# Autodesk Inventor assembly: Pick_&_Place_Nozzle_Assembly
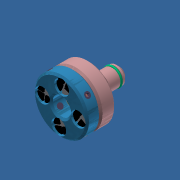
[picture p0: Inventor's stored thumbnail of the model, 180x180]
Saved by Autodesk Inventor 2015 (Build 190159000, 159)
## iProperties
Created: 2015-01-06
Part Number: Pick_&_Place_Nozzle_Assembly
Document SubType Name: Assembly
Designer: ice
Author: ice
## Documents named in this file (8)
- C:\Users\ice\Documents\GitHub\PnP-Magnetic-Tool-Tip\Inventor\Extender_Assembly_Rev_C.iam
- C:\Users\ice\Documents\GitHub\PnP-Magnetic-Tool-Tip\Inventor\Magnet_Extender_Split_Top_Rev_C.ipt
- C:\Users\ice\Documents\GitHub\PnP-Magnetic-Tool-Tip\Inventor\Magnet_Extender_Split_Bottom_Rev_C.ipt
- C:\Users\ice\Documents\GitHub\PnP-Magnetic-Tool-Tip\Inventor\o_ring_5.00_0.5.ipt
- C:\Users\ice\Documents\GitHub\PnP-Magnetic-Tool-Tip\Inventor\M1.6x5_Headless.ipt
- C:\Users\ice\Documents\GitHub\PnP-Magnetic-Tool-Tip\Inventor\M2x5_D963.ipt
- C:\Users\ice\Documents\GitHub\PnP-Magnetic-Tool-Tip\Inventor\o_ring_4.29_0.5XXX.ipt
- C:\Users\ice\Documents\GitHub\PnP-Magnetic-Tool-Tip\Inventor\Magnet10x1x5.ipt
## Components (14 placed, 7 different names)
1. Magnet_Extender_Split_Top_Rev_C:1 — Mate:1, Mate:2, Mate:3, Mate:5, Mate:20, Mate:21, Mate:22, Flush:3, Mate:23, Flush:4
2. Magnet_Extender_Split_Bottom_Rev_C:1 — Mate:1, Mate:2, Mate:3, Mate:4, Mate:6, Mate:7, Mate:8, Mate:9, Flush:1, Mate:10, Mate:11, Flush:2, Mate:12, Mate:13, Mate:14, Mate:15, Mate:16, Mate:17, Mate:18, Mate:19
3. o_ring_5.00_0.5:1 — Mate:4, Mate:5
4. M1.6x5_Headless:1 — Mate:6, Mate:10
5. M1.6x5_Headless:2 — Mate:7, Flush:2
6. M1.6x5_Headless:3 — Mate:8, Flush:1
7. M1.6x5_Headless:4 — Mate:9, Mate:11
8. M2x5_D963:1 — Mate:12, Mate:19
9. M2x5_D963:2 — Mate:13, Mate:18
10. M2x5_D963:3 — Mate:14, Mate:17
11. M2x5_D963:4 — Mate:15, Mate:16
12. o_ring_4.29_0.5XXX:1 — Mate:20, Flush:3
13. o_ring_4.29_0.5XXX:2 — Mate:21, Mate:22
14. Magnet10x1x5:1 — Mate:23, Flush:4
## Relationships (27: Mate 23, Flush 4)
- Mate:1: Magnet_Extender_Split_Top_Rev_C:1 ↔ Magnet_Extender_Split_Bottom_Rev_C:1
- Mate:2: Magnet_Extender_Split_Top_Rev_C:1 ↔ Magnet_Extender_Split_Bottom_Rev_C:1
- Mate:3: Magnet_Extender_Split_Top_Rev_C:1 ↔ Magnet_Extender_Split_Bottom_Rev_C:1
- Mate:4: Magnet_Extender_Split_Bottom_Rev_C:1 ↔ o_ring_5.00_0.5:1
- Mate:5: Magnet_Extender_Split_Top_Rev_C:1 ↔ o_ring_5.00_0.5:1
- Mate:6: Magnet_Extender_Split_Bottom_Rev_C:1 ↔ M1.6x5_Headless:1
- Mate:7: Magnet_Extender_Split_Bottom_Rev_C:1 ↔ M1.6x5_Headless:2
- Mate:8: Magnet_Extender_Split_Bottom_Rev_C:1 ↔ M1.6x5_Headless:3
- Mate:9: Magnet_Extender_Split_Bottom_Rev_C:1 ↔ M1.6x5_Headless:4
- Flush:1: Magnet_Extender_Split_Bottom_Rev_C:1 ↔ M1.6x5_Headless:3
- Mate:10: Magnet_Extender_Split_Bottom_Rev_C:1 ↔ M1.6x5_Headless:1
- Mate:11: Magnet_Extender_Split_Bottom_Rev_C:1 ↔ M1.6x5_Headless:4
- Flush:2: Magnet_Extender_Split_Bottom_Rev_C:1 ↔ M1.6x5_Headless:2
- Mate:12: Magnet_Extender_Split_Bottom_Rev_C:1 ↔ M2x5_D963:1
- Mate:13: Magnet_Extender_Split_Bottom_Rev_C:1 ↔ M2x5_D963:2
- Mate:14: Magnet_Extender_Split_Bottom_Rev_C:1 ↔ M2x5_D963:3
- Mate:15: Magnet_Extender_Split_Bottom_Rev_C:1 ↔ M2x5_D963:4
- Mate:16: Magnet_Extender_Split_Bottom_Rev_C:1 ↔ M2x5_D963:4
- Mate:17: Magnet_Extender_Split_Bottom_Rev_C:1 ↔ M2x5_D963:3
- Mate:18: Magnet_Extender_Split_Bottom_Rev_C:1 ↔ M2x5_D963:2
- Mate:19: Magnet_Extender_Split_Bottom_Rev_C:1 ↔ M2x5_D963:1
- Mate:20: Magnet_Extender_Split_Top_Rev_C:1 ↔ o_ring_4.29_0.5XXX:1
- Mate:21: Magnet_Extender_Split_Top_Rev_C:1 ↔ o_ring_4.29_0.5XXX:2
- Mate:22: Magnet_Extender_Split_Top_Rev_C:1 ↔ o_ring_4.29_0.5XXX:2
- Flush:3: Magnet_Extender_Split_Top_Rev_C:1 ↔ o_ring_4.29_0.5XXX:1
- Mate:23: Magnet_Extender_Split_Top_Rev_C:1 ↔ Magnet10x1x5:1
- Flush:4: Magnet_Extender_Split_Top_Rev_C:1 ↔ Magnet10x1x5:1
